# Autodesk Inventor assembly: motor_plant_assembly
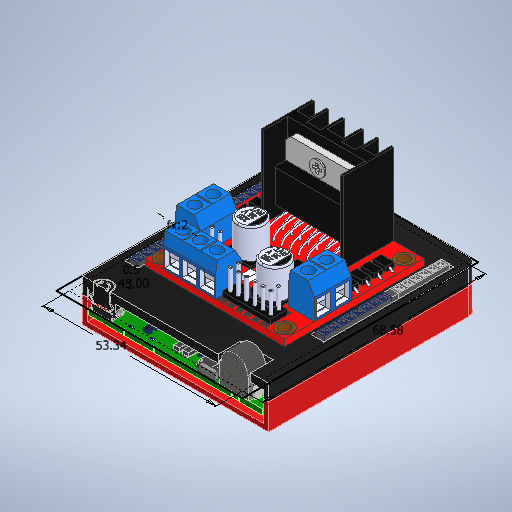
[picture p0: Inventor's stored thumbnail of the model, 512x512]
Saved by Autodesk Inventor 2025.2 (Build 292293000, 293)
## iProperties
Created: 2025-03-24
Part Number: motor_plant_assembly
Document SubType Name: Assembly
Designer: caomi
Author: caomi
## Documents named in this file (5)
- C:\mnguyen\small-controls-project\cad\motor_plant_assembly.iam
- C:\mnguyen\small-controls-project\cad\uno_r4_base.ipt
- C:\mnguyen\small-controls-project\cad\uno_r4_minima.iam
- C:\mnguyen\small-controls-project\cad\uno_r4_lid.ipt
- C:\mnguyen\small-controls-project\cad\L298N Driver DC Motor, Stepper Motor.ipt
## Components (4 placed, 4 different names)
1. uno_r4_base:1 — Rigid:1, Rigid:2
2. uno_r4_minima:1 [sub-assembly] — Rigid:1
3. uno_r4_lid:1 — Rigid:2, Rigid:3
4. L298N Driver DC Motor, Stepper Motor:1 — Rigid:3
## Relationships (3: WeldJoint 3)
- Rigid:1 [WeldJoint]: uno_r4_base:1 ↔ uno_r4_minima:1
- Rigid:2 [WeldJoint]: uno_r4_base:1 ↔ uno_r4_lid:1
- Rigid:3 [WeldJoint]: uno_r4_lid:1 ↔ L298N Driver DC Motor, Stepper Motor:1
